# Autodesk Inventor assembly: Assembly1
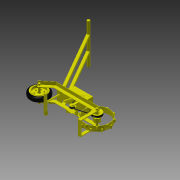
[picture p0: Inventor's stored thumbnail of the model, 180x180]
Saved by Autodesk Inventor 2015 (Build 190159000, 159)
## iProperties
Created: 2015-09-11
Part Number: Assembly1
Document SubType Name: Assembly
Designer: Okorie Ifeanyichukwu
Author: Okorie Ifeanyichukwu
## Documents named in this file (7)
- C:\Users\Okorie Ifeanyichukwu\Documents\inventor\Nnamdi\Assembly1.iam
- C:\Users\Okorie Ifeanyichukwu\Documents\inventor\Nnamdi\frame.ipt
- C:\Users\Okorie Ifeanyichukwu\Documents\inventor\Nnamdi\front.ipt
- C:\Users\Okorie Ifeanyichukwu\Documents\inventor\Nnamdi\hopper.ipt
- C:\Users\Okorie Ifeanyichukwu\Documents\inventor\Nnamdi\rear.ipt
- C:\Users\Okorie Ifeanyichukwu\Documents\inventor\Nnamdi\shaft.ipt
- C:\Users\Okorie Ifeanyichukwu\Documents\inventor\Nnamdi\Assembly1\Design Accelerator\V-Belt transmission1.iam
## Components (6 placed, 6 different names)
1. frame:1 — Insert:1, Mate:1, Insert:2
2. front:1 — Insert:1
3. hopper:1 — Mate:1, Insert:3
4. rear:1 — Insert:2
5. shaft:1 — Insert:3
6. V-Belt transmission:1 [sub-assembly]
## Relationships (4: Insert 3, Mate 1)
- Insert:1 (60 mm): frame:1 ↔ front:1
- Mate:1: frame:1 ↔ hopper:1
- Insert:2 (90 mm): frame:1 ↔ rear:1
- Insert:3 (30 mm): hopper:1 ↔ shaft:1
